# Autodesk Inventor assembly: Osnovanie
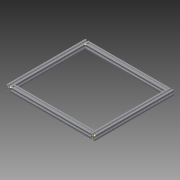
[picture p0: Inventor's stored thumbnail of the model, 180x180]
Saved by Autodesk Inventor 2015 (Build 190159000, 159)
## iProperties
Created: 2016-04-26
Part Number: Osnovanie
Document SubType Name: Assembly
Designer: Andreas
Author: Andreas
## Documents named in this file (2)
- C:\Users\Andreas\Desktop\Osnovanie.iam
- C:\Users\Andreas\Documents\Inventor\Balka.ipt
## Components (4 placed, 1 different names)
1. Balka:1 — Rigid:1, Rigid:2
2. Balka:2 — Rigid:1, Rigid:3
3. Balka:3 — Rigid:3
4. Balka:4 — Rigid:2
## Relationships (3: WeldJoint 3)
- Rigid:1 [WeldJoint]: Balka:1 ↔ Balka:2
- Rigid:2 [WeldJoint]: Balka:1 ↔ Balka:4
- Rigid:3 [WeldJoint]: Balka:2 ↔ Balka:3
